# Autodesk Inventor assembly: Assembly5 NEW
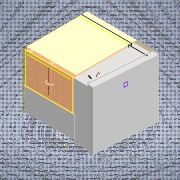
[picture p0: Inventor's stored thumbnail of the model, 180x180]
Saved by Autodesk Inventor 2021 (Build 250183000, 183)
## iProperties
Created: 2021-07-27
Part Number: Assembly5 NEW
Document SubType Name: Assembly
Designer: Bharath Koli
Author: Bharath Koli
## Documents named in this file (8)
- E:\engg\SMARTLOCKER\Assembly5 NEW.iam
- E:\engg\SMARTLOCKER\NEW.ipt
- E:\engg\SMARTLOCKER\PLACER 1.ipt
- E:\engg\SMARTLOCKER\DC Motor (1).ipt
- E:\engg\SMARTLOCKER\Assembly78.iam
- E:\engg\SMARTLOCKER\Servomotor HTX900 set new 3.iam
- E:\engg\SMARTLOCKER\NEW PART 2.ipt
- E:\engg\SMARTLOCKER\Part1nrt.ipt
## Components (7 placed, 7 different names)
1. NEW:1 — Mate:1
2. PLACER 1:1
3. DC Motor (1):1
4. Assembly78:1 [sub-assembly] — Mate:1
5. Servomotor HTX900 set new 3:1 [sub-assembly]
6. NEW PART 2:1
7. Part1nrt:1
## Relationships (1: Mate 1)
- Mate:1: NEW:1 ↔ Assembly78:1
